# Autodesk Inventor assembly: 100mmActuator
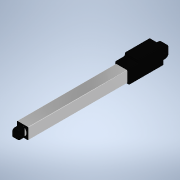
[picture p0: Inventor's stored thumbnail of the model, 180x180]
Saved by Autodesk Inventor 2020 (Build 240168000, 168)
## iProperties
Created: 2023-02-03
Part Number: 100mmActuator
Document SubType Name: Assembly
Designer: legoo
Author: legoo
## Documents named in this file (3)
- C:\Users\Public\Documents\Autodesk\Inventor 2020\projects\3156\actuators\100mmActuator.iam
- C:\Users\Public\Documents\Autodesk\Inventor 2020\projects\3156\actuators\100mmStrokeBase.ipt
- C:\Users\Public\Documents\Autodesk\Inventor 2020\projects\3156\actuators\100mmStrokeRod.ipt
## Components (2 placed, 2 different names)
1. 100mmStrokeBase:1 — Mate:1, Angle:1, Flush:1, Mate:2, Mate:3
2. 100mmStrokeRod:1 — Mate:1, Angle:1
## Relationships (5: Mate 3, Angle 1, Flush 1)
- Mate:1: 100mmStrokeBase:1 ↔ 100mmStrokeRod:1
- Angle:1 (0 deg): 100mmStrokeBase:1 ↔ 100mmStrokeRod:1
- Flush:1: 100mmStrokeBase:1
- Mate:2: 100mmStrokeBase:1
- Mate:3: 100mmStrokeBase:1
